# Autodesk Inventor assembly: Gantry Side load assy
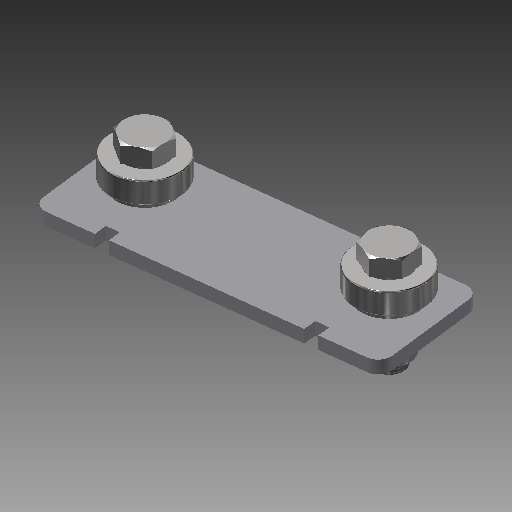
[picture p0: Inventor's stored thumbnail of the model, 512x512]
Saved by Autodesk Inventor 2018.2 (Build 222227000, 227)
## iProperties
Created: 2017-12-19
Part Number: Gantry Side load assy
Document SubType Name: Assembly
Designer: torba
Author: torba
## Documents named in this file (3)
- C:\Users\torba\OneDrive\Documents\Inventor\Plasma 5x10\Gantry Side load assy.iam
- C:\Users\torba\OneDrive\Documents\Inventor\Plasma 5x10\Gantry side load.ipt
- C:\Users\torba\OneDrive\Documents\Inventor\Plasma 5x10\Bearing Assembly.iam
## Components (3 placed, 2 different names)
1. Gantry side load:1 — Mate:1, Mate:2, Mate:3, Mate:4
2. Bearing Assembly:1 [sub-assembly] — Mate:2, Mate:4
3. Bearing Assembly:2 [sub-assembly] — Mate:1, Mate:3
## Relationships (4: Mate 4)
- Mate:1: Gantry side load:1 ↔ Bearing Assembly:2
- Mate:2: Gantry side load:1 ↔ Bearing Assembly:1
- Mate:3: Gantry side load:1 ↔ Bearing Assembly:2
- Mate:4: Gantry side load:1 ↔ Bearing Assembly:1
